# Autodesk Inventor assembly: s-assy-gripper_tentioner
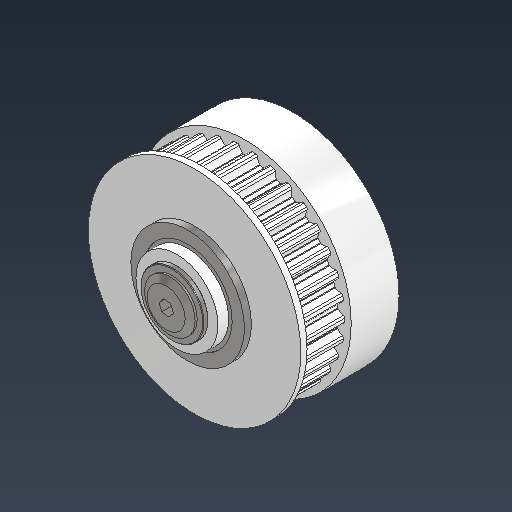
[picture p0: Inventor's stored thumbnail of the model, 512x512]
Saved by Autodesk Inventor 2021 (Build 250183000, 183)
## iProperties
Created: 2021-08-06
Part Number: s-assy-gripper_tentioner
Document SubType Name: Assembly
Designer: yuta0
Mass: 598.977 g
Surface Area: 2161.2 cm^2
Volume: 259.929 cm^3
Density: 2.30439 g/cm^3
Author: yuta0
## Documents named in this file (9)
- C:\Users\yuta0\Documents\GitHub\catchrobo_hardware\assy-robot\s-assy-gripper_tentioner.iam
- C:\Users\yuta0\Documents\GitHub\catchrobo_hardware\assy-robot\base36.ipt
- C:\Users\yuta0\Documents\GitHub\catchrobo_hardware\assy-robot\FL688ZZ.ipt
- C:\Users\yuta0\Documents\GitHub\catchrobo_hardware\assy-robot\CB4-6.ipt
- C:\Users\yuta0\Documents\GitHub\catchrobo_hardware\assy-robot\CC-0814-05.ipt
- C:\Users\yuta0\Documents\GitHub\catchrobo_hardware\assy-robot\ARF-420E.ipt
- C:\Users\yuta0\Documents\GitHub\catchrobo_hardware\assy-robot\WSJ-STN-M4.ipt
- C:\Users\yuta0\Documents\GitHub\catchrobo_hardware\assy-robot\base39.ipt
- C:\Users\yuta0\Documents\GitHub\catchrobo_hardware\assy-robot\CBSTSR4-6.ipt
## Components (10 placed, 8 different names)
1. ARF-420E:1 — メイト:78, メイト:80, メイト:81, メイト:86, メイト:94, メイト:123
2. CC-0814-05:1 — メイト:38, メイト:39, メイト:125
3. FL688ZZ:2 — メイト:29, メイト:30, メイト:39
4. WSJ-STN-M4:2 — メイト:87, メイト:125, メイト:127
5. CB4-6:8 — メイト:86, メイト:87
6. CBSTSR4-6:3 — メイト:123, メイト:124
7. WSJ-STN-M4:1 — メイト:80, メイト:81, メイト:124, メイト:126
8. base39:1 — メイト:94, メイト:95, メイト:126
9. FL688ZZ:1 — メイト:26, メイト:28, メイト:38, メイト:78, メイト:95
10. base36:1 — メイト:26, メイト:28, メイト:29, メイト:30, メイト:127
## Relationships (18: Mate 18)
- メイト:26 [Mate]: FL688ZZ:1 ↔ base36:1
- メイト:28 [Mate]: FL688ZZ:1 ↔ base36:1
- メイト:29 [Mate]: FL688ZZ:2 ↔ base36:1
- メイト:30 [Mate]: FL688ZZ:2 ↔ base36:1
- メイト:38 [Mate]: CC-0814-05:1 ↔ FL688ZZ:1
- メイト:39 [Mate]: CC-0814-05:1 ↔ FL688ZZ:2
- メイト:78 [Mate]: ARF-420E:1 ↔ FL688ZZ:1
- メイト:80 [Mate]: ARF-420E:1 ↔ WSJ-STN-M4:1
- メイト:81 [Mate]: ARF-420E:1 ↔ WSJ-STN-M4:1
- メイト:86 [Mate]: ARF-420E:1 ↔ CB4-6:8
- メイト:87 [Mate]: WSJ-STN-M4:2 ↔ CB4-6:8
- メイト:94 [Mate]: ARF-420E:1 ↔ base39:1
- メイト:95 [Mate]: base39:1 ↔ FL688ZZ:1
- メイト:123 [Mate]: ARF-420E:1 ↔ CBSTSR4-6:3
- メイト:124 [Mate]: CBSTSR4-6:3 ↔ WSJ-STN-M4:1
- メイト:125 [Mate] (2 mm): CC-0814-05:1 ↔ WSJ-STN-M4:2
- メイト:126 [Mate]: WSJ-STN-M4:1 ↔ base39:1
- メイト:127 [Mate]: WSJ-STN-M4:2 ↔ base36:1
